# Autodesk Inventor assembly: ASY GBK правая стенка
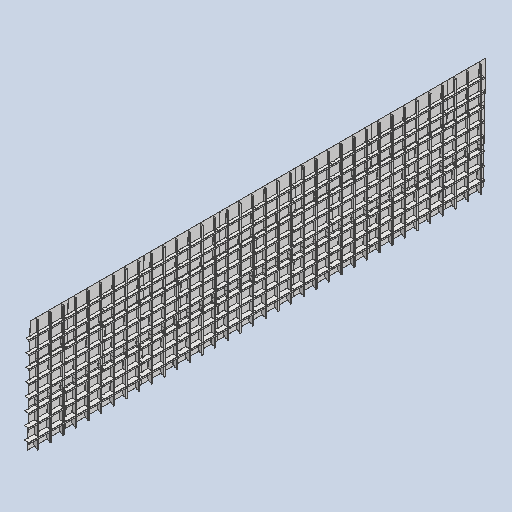
[picture p0: Inventor's stored thumbnail of the model, 512x512]
Saved by Autodesk Inventor 2026 (Build 300175000, 175)
## iProperties
Created: 2026-05-20
Part Number: ASY GBK правая стенка
Document SubType Name: Assembly
Designer: admin
Mass: 4.44159e+06 g
Surface Area: 2.86879e+06 cm^2
Volume: 565808 cm^3
Density: 7.85 g/cm^3
Author: admin
## Documents named in this file (6)
- C:\Users\pokla\Documents\Inventor\GBK-Gubkinskiy\ASY GBK правая стенка.iam
- C:\Users\pokla\Documents\Inventor\GBK-Gubkinskiy\ASY GBK 1110 long wall shield 1.iam
- C:\Users\pokla\Documents\Inventor\GBK-Gubkinskiy\ASY GBK 1120 long wall shield 2.iam
- C:\Users\pokla\Documents\Inventor\GBK-Gubkinskiy\ASY GBK 1210 long wall shield 3.iam
- C:\Users\pokla\Documents\Inventor\GBK-Gubkinskiy\ASY GBK 1310 long wall shield 4.iam
- C:\Users\pokla\Documents\Inventor\GBK-Gubkinskiy\ASY GBK 1320 long wall shield 5.iam
## Components (20 placed, 5 different names)
1. ASY GBK 1110 long wall shield 1.iam:1 [sub-assembly] — Заподлицо:1, Совмещение:1, Совмещение:2
2. ASY GBK 1120 long wall shield 2.iam:1 [sub-assembly]
3. ASY GBK 1210 long wall shield 3.iam:1 [sub-assembly]
4. ASY GBK 1310 long wall shield 4.iam:1 [sub-assembly]
5. ASY GBK 1320 long wall shield 5.iam:1 [sub-assembly]
6. ASY GBK 1320 long wall shield 5.iam:2 [sub-assembly]
7. ASY GBK 1320 long wall shield 5.iam:3 [sub-assembly]
8. ASY GBK 1320 long wall shield 5.iam:4 [sub-assembly]
9. ASY GBK 1320 long wall shield 5.iam:5 [sub-assembly]
10. ASY GBK 1210 long wall shield 3.iam:2 [sub-assembly]
11. ASY GBK 1210 long wall shield 3.iam:3 [sub-assembly]
12. ASY GBK 1210 long wall shield 3.iam:4 [sub-assembly]
13. ASY GBK 1210 long wall shield 3.iam:5 [sub-assembly]
14. ASY GBK 1210 long wall shield 3.iam:6 [sub-assembly]
15. ASY GBK 1120 long wall shield 2.iam:2 [sub-assembly]
16. ASY GBK 1120 long wall shield 2.iam:3 [sub-assembly]
17. ASY GBK 1120 long wall shield 2.iam:4 [sub-assembly]
18. ASY GBK 1120 long wall shield 2.iam:5 [sub-assembly]
19. ASY GBK 1110 long wall shield 1.iam:2 [sub-assembly]
20. ASY GBK 1310 long wall shield 4.iam:2 [sub-assembly]
## Relationships (22: WeldJoint 19, Mate 2, Flush 1)
- [WeldJoint] (1 mm): ASY GBK 1110 long wall shield 1.iam:1 ↔ ASY GBK 1120 long wall shield 2.iam:1
- [WeldJoint]: ASY GBK 1110 long wall shield 1.iam:1 ↔ ASY GBK 1210 long wall shield 3.iam:1
- [WeldJoint]: ASY GBK 1210 long wall shield 3.iam:1 ↔ ASY GBK 1310 long wall shield 4.iam:1
- [WeldJoint] (1 mm): ASY GBK 1310 long wall shield 4.iam:1 ↔ ASY GBK 1320 long wall shield 5.iam:1
- [WeldJoint] (1 mm): ASY GBK 1320 long wall shield 5.iam:1 ↔ ASY GBK 1320 long wall shield 5.iam:2
- [WeldJoint] (1 mm): ASY GBK 1320 long wall shield 5.iam:2 ↔ ASY GBK 1320 long wall shield 5.iam:3
- [WeldJoint] (1 mm): ASY GBK 1320 long wall shield 5.iam:3 ↔ ASY GBK 1320 long wall shield 5.iam:4
- [WeldJoint] (1 mm): ASY GBK 1320 long wall shield 5.iam:4 ↔ ASY GBK 1320 long wall shield 5.iam:5
- [WeldJoint] (1 mm): ASY GBK 1210 long wall shield 3.iam:1 ↔ ASY GBK 1210 long wall shield 3.iam:2
- [WeldJoint] (1 mm): ASY GBK 1210 long wall shield 3.iam:2 ↔ ASY GBK 1210 long wall shield 3.iam:3
- [WeldJoint] (1 mm): ASY GBK 1210 long wall shield 3.iam:3 ↔ ASY GBK 1210 long wall shield 3.iam:4
- [WeldJoint] (1 mm): ASY GBK 1210 long wall shield 3.iam:4 ↔ ASY GBK 1210 long wall shield 3.iam:5
- [WeldJoint] (1 mm): ASY GBK 1210 long wall shield 3.iam:5 ↔ ASY GBK 1210 long wall shield 3.iam:6
- [WeldJoint] (1 mm): ASY GBK 1120 long wall shield 2.iam:1 ↔ ASY GBK 1120 long wall shield 2.iam:2
- [WeldJoint] (1 mm): ASY GBK 1120 long wall shield 2.iam:2 ↔ ASY GBK 1120 long wall shield 2.iam:3
- [WeldJoint] (1 mm): ASY GBK 1120 long wall shield 2.iam:3 ↔ ASY GBK 1120 long wall shield 2.iam:4
- [WeldJoint] (1 mm): ASY GBK 1120 long wall shield 2.iam:4 ↔ ASY GBK 1120 long wall shield 2.iam:5
- [WeldJoint] (1 mm): ASY GBK 1120 long wall shield 2.iam:5 ↔ ASY GBK 1110 long wall shield 1.iam:2
- [WeldJoint] (1 mm): ASY GBK 1320 long wall shield 5.iam:5 ↔ ASY GBK 1310 long wall shield 4.iam:2
- Заподлицо:1 [Flush]: ASY GBK 1110 long wall shield 1.iam:1
- Совмещение:1 [Mate]: ASY GBK 1110 long wall shield 1.iam:1
- Совмещение:2 [Mate]: ASY GBK 1110 long wall shield 1.iam:1
## Named parameters: Зазор_по_горизонту = 1 mm
